# Autodesk Inventor assembly: Arm
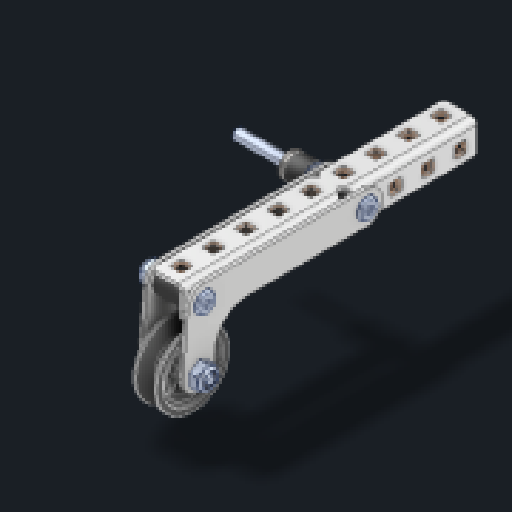
[picture p0: Inventor's stored thumbnail of the model, 512x512]
Saved by Autodesk Inventor 2025.1 (Build 291241000, 241)
## iProperties
Created: 2024-10-24
Part Number: Arm
Document SubType Name: Assembly
Designer: avere
Author: avere
## Documents named in this file (16)
- C:\Users\avere\VEX\High Stakes\CAD\V2\Hang\Arm.iam
- C:\Users\avere\VEX\High Stakes\CAD\ROBOPROS-CAD-Inventor\Structure\Angle\Aluminum 1x1\Alu Angle 1x1x9.ipt
- C:\Users\avere\VEX\High Stakes\CAD\ROBOPROS-CAD-Inventor\Motion\Spacers\Spacer Nylon .375 OD\NSpacer .375 OD x .500.ipt
- C:\Users\avere\VEX\High Stakes\CAD\ROBOPROS-CAD-Inventor\Motion\Spacers\Spacer Nylon .375 OD.ipt
- C:\Users\avere\VEX\High Stakes\CAD\V2\Hang\Custom Parts\Passive Gusset.ipt
- C:\Users\avere\VEX\High Stakes\CAD\ROBOPROS-CAD-Inventor\Motion\Pulley.ipt
- C:\Users\avere\VEX\High Stakes\CAD\ROBOPROS-CAD-Inventor\Structure\Hardware\Nut Keps.ipt
- C:\Users\avere\VEX\High Stakes\CAD\ROBOPROS-CAD-Inventor\Structure\Hardware\Screw Shoulder Robosource\SScrew Shoulder Smooth 2.000 x .04.ipt
- C:\Users\avere\VEX\High Stakes\CAD\ROBOPROS-CAD-Inventor\Structure\Hardware\Screw Shoulder Robosource.ipt
- C:\Users\avere\VEX\High Stakes\CAD\ROBOPROS-CAD-Inventor\Motion\Spacers\Spacer Nylon .375 OD\NSpacer .375 OD x .250.ipt
- C:\Users\avere\VEX\High Stakes\CAD\ROBOPROS-CAD-Inventor\Motion\Spacers\Washer Steel\SWasher .375 OD x .031250.ipt
- C:\Users\avere\VEX\High Stakes\CAD\ROBOPROS-CAD-Inventor\Motion\Spacers\Washer Steel.ipt
- C:\Users\avere\VEX\High Stakes\CAD\ROBOPROS-CAD-Inventor\Motion\Spacers\Washer Steel\SWasher .375 OD x .062500.ipt
- C:\Users\avere\VEX\High Stakes\CAD\ROBOPROS-CAD-Inventor\Structure\Hardware\Screw Steel - Star\SScrew Star Smooth .875.ipt
- C:\Users\avere\VEX\High Stakes\CAD\ROBOPROS-CAD-Inventor\Structure\Hardware\Screw Steel - Star.ipt
- C:\Users\avere\VEX\High Stakes\CAD\ROBOPROS-CAD-Inventor\Structure\Hardware\Nut Thin Nylock.ipt
## Components (16 placed, 11 different names)
1. Alu Angle 1x1x9:1 — Insert:1, Insert:2, Insert:3, Mate:1
2. NSpacer .375 OD x .500:1 — Insert:2, Mate:2
3. NSpacer .375 OD x .500:2 — Insert:1, Insert:4
4. Passive Gusset:1 — Insert:3, Mate:1, Insert:8, Insert:12, Insert:14
5. Passive Gusset:2 — Insert:4, Mate:2, Insert:5, Insert:7, Insert:13, Insert:15
6. Pulley:1 — Insert:6
7. Nut Keps:1 — Insert:5, Insert:6
8. Nut Keps:2 — Insert:7, Insert:11
9. SScrew Shoulder Smooth 2.000 x .04:1 — Insert:8
10. NSpacer .375 OD x .250:3 — Insert:9, Insert:11
11. SWasher .375 OD x .031250:1 — Insert:10
12. SWasher .375 OD x .062500:2 — Insert:9, Insert:10
13. SScrew Star Smooth .875:1 — Insert:12
14. Nut Thin Nylock:1 — Insert:13
15. Nut Thin Nylock:2 — Insert:14
16. SScrew Star Smooth .875:2 — Insert:15
## Relationships (17: Insert 15, Mate 2)
- Insert:1: Alu Angle 1x1x9:1 ↔ NSpacer .375 OD x .500:2
- Insert:2: Alu Angle 1x1x9:1 ↔ NSpacer .375 OD x .500:1
- Insert:3: Alu Angle 1x1x9:1 ↔ Passive Gusset:1
- Mate:1: Alu Angle 1x1x9:1 ↔ Passive Gusset:1
- Insert:4: NSpacer .375 OD x .500:2 ↔ Passive Gusset:2
- Mate:2: NSpacer .375 OD x .500:1 ↔ Passive Gusset:2
- Insert:5: Passive Gusset:2 ↔ Nut Keps:1
- Insert:6 (0.3969 mm): Pulley:1 ↔ Nut Keps:1
- Insert:7: Passive Gusset:2 ↔ Nut Keps:2
- Insert:8: Passive Gusset:1 ↔ SScrew Shoulder Smooth 2.000 x .04:1
- Insert:9: NSpacer .375 OD x .250:3 ↔ SWasher .375 OD x .062500:2
- Insert:10: SWasher .375 OD x .031250:1 ↔ SWasher .375 OD x .062500:2
- Insert:11: Nut Keps:2 ↔ NSpacer .375 OD x .250:3
- Insert:12: Passive Gusset:1 ↔ SScrew Star Smooth .875:1
- Insert:13: Passive Gusset:2 ↔ Nut Thin Nylock:1
- Insert:14: Passive Gusset:1 ↔ Nut Thin Nylock:2
- Insert:15: Passive Gusset:2 ↔ SScrew Star Smooth .875:2
